# Autodesk Inventor assembly: axis
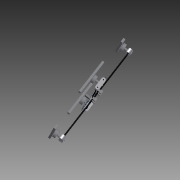
[picture p0: Inventor's stored thumbnail of the model, 180x180]
Saved by Autodesk Inventor 2013 (Build 170138000, 138)
## iProperties
Created: 2013-01-16
Part Number: axis
Document SubType Name: Assembly
Designer: geohot
Author: geohot
## Documents named in this file (5)
- C:\Users\geohot\Documents\GitHub\quadrotor\cad\axis.iam
- C:\Users\geohot\Documents\GitHub\quadrotor\cad\motor.iam
- C:\Users\geohot\Documents\GitHub\quadrotor\cad\rod.ipt
- C:\Users\geohot\Documents\GitHub\quadrotor\cad\quad.ipt
- C:\Users\geohot\Documents\GitHub\quadrotor\cad\Imported Components\daboard\daboard.iam
## Components (13 placed, 4 different names)
1. rod:1 — Insert:11, Insert:13, Mate:16, Mate:17
2. rod:2 — Mate:14, Insert:12, Insert:14, Mate:21
3. motor:3 [sub-assembly] — Insert:5, Insert:6, Mate:10
4. motor:4 [sub-assembly] — Insert:7, Insert:8
5. rod:3 — Insert:5, Insert:7, Mate:15, Mate:23
6. rod:4 — Insert:6, Insert:8, Mate:18, Mate:20
7. quad:4 — Mate:10, Mate:14, Mate:23, Insert:15
8. motor:6 [sub-assembly] — Insert:11, Insert:12
9. motor:7 [sub-assembly] — Insert:13, Insert:14, Mate:22
10. quad:5 — Mate:15, Mate:16, Mate:22
11. quad:6 — Mate:17, Mate:18, Mate:19, Insert:16
12. quad:7 — Mate:19, Mate:20, Mate:21
13. daboard:1 [sub-assembly] — Insert:15, Insert:16
## Relationships (21: Mate 11, Insert 10)
- Insert:5: motor:3 ↔ rod:3
- Insert:6: motor:3 ↔ rod:4
- Insert:7: motor:4 ↔ rod:3
- Insert:8: motor:4 ↔ rod:4
- Mate:10 (123.825 mm): motor:3 ↔ quad:4
- Mate:14: rod:2 ↔ quad:4
- Insert:11: rod:1 ↔ motor:6
- Insert:12: rod:2 ↔ motor:6
- Insert:13: rod:1 ↔ motor:7
- Insert:14: rod:2 ↔ motor:7
- Mate:15: rod:3 ↔ quad:5
- Mate:16: rod:1 ↔ quad:5
- Mate:17: rod:1 ↔ quad:6
- Mate:18: rod:4 ↔ quad:6
- Mate:19 (19.05 mm): quad:6 ↔ quad:7
- Mate:20: rod:4 ↔ quad:7
- Mate:21: rod:2 ↔ quad:7
- Mate:22 (123.825 mm): motor:7 ↔ quad:5
- Mate:23: rod:3 ↔ quad:4
- Insert:15: quad:4 ↔ daboard:1
- Insert:16: quad:6 ↔ daboard:1
